# Autodesk Inventor assembly: 2020RobotV3
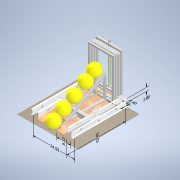
[picture p0: Inventor's stored thumbnail of the model, 180x180]
Saved by Autodesk Inventor 2020.2 (Build 242310000, 310)
## iProperties
Created: 2020-01-12
Part Number: 2020RobotV3
Document SubType Name: Assembly
Designer: robst
Author: robst
## Documents named in this file (15)
- C:\git\CAD-Development\robSteele\2020LongRobotBase\2020RobotV3.iam
- C:\git\CAD-Development\robSteele\2020LongRobotBase\2020 Wood Base.ipt
- C:\git\CAD-Development\robSteele\2020LongRobotBase\2020 End Plate.ipt
- C:\git\CAD-Development\robSteele\2020LongRobotBase\am-3921 AM14U4 Outside Plate.ipt
- C:\git\CAD-Development\robSteele\2020LongRobotBase\am-3922 AM14U4 Inside Plate.ipt
- C:\git\CAD-Development\robSteele\2020LongRobotBase\crossPlate.ipt
- C:\git\CAD-Development\robSteele\2020LongRobotBase\floor.ipt
- C:\git\CAD-Development\robSteele\2020LongRobotBase\1892-YEL.ipt
- C:\git\CAD-Development\robSteele\2020LongRobotBase\ceiling.ipt
- C:\git\CAD-Development\robSteele\2020LongRobotBase\asPrototypedBallRamp.iam
- C:\git\CAD-Development\robSteele\2020LongRobotBase\asPrototypedBallRamp_MIR.iam
- C:\git\CAD-Development\robSteele\2020LiftMechanism\primativeBaseForShortRobot.ipt
- C:\git\CAD-Development\robSteele\2020LiftMechanism\primative1stStageForShortRobot.ipt
- C:\git\CAD-Development\robSteele\2020LiftMechanism\primative4thStageForShortRobot.ipt
- C:\git\CAD-Development\robSteele\2020LiftMechanism\primative3rdStageForShortRobot.ipt
## Components (20 placed, 14 different names)
1. 2020 End Plate:1 — Mate:2, Mate:3, Mate:5, Mate:6, Flush:2, Flush:3, Mate:7, Mate:8, Mate:13, Mate:14, Mate:33, Flush:14, Mate:42, Mate:68
2. am-3921 AM14U4 Outside Plate:1 — Mate:5, Mate:6, Flush:2, Mate:15
3. am-3921 AM14U4 Outside Plate:2 — Mate:2, Mate:3, Flush:3, Mate:9
4. am-3922 AM14U4 Inside Plate:1 — Mate:7, Mate:8, Mate:9, Mate:12, Flush:4, Flush:5, Flush:12, Mate:32
5. crossPlate:1 — Mate:12, Flush:4, Flush:5
6. am-3922 AM14U4 Inside Plate:2 — Mate:13, Mate:14, Mate:15
7. floor:1 — Mate:54, Mate:55, Flush:18, Mate:65, Mate:66, Flush:30
8. 1892-YEL:1 — Mate:46, Mate:51
9. 1892-YEL:2 — Mate:50, Mate:52
10. 1892-YEL:3 — Mate:47, Mate:53
11. 1892-YEL:4 — Mate:48
12. 1892-YEL:5 — Mate:49
13. ceiling:1 — Mate:65, Mate:66, Flush:30
14. 2020 Wood Base:1 — Flush:13, Mate:32, Mate:33, Mate:35, Mate:37, Flush:16, Mate:39, Mate:54
15. asPrototypedBallRamp:1 [sub-assembly] — Mate:34, Mate:35, Flush:14, Flush:17
16. asPrototypedBallRamp_MIR:1 [sub-assembly] — Flush:15
17. primativeBaseForShortRobot:1 — Mate:36, Mate:37, Flush:16, Mate:40
18. primative1stStageForShortRobot:1 — Mate:38, Mate:39, Mate:40, Mate:43
19. primative3rdStageForShortRobot:1 — Mate:41, Mate:42, Mate:43, Mate:45
20. primative4thStageForShortRobot:1 — Mate:45, Mate:67, Mate:68
## Relationships (50: Mate 38, Flush 12)
- Mate:2: 2020 End Plate:1 ↔ am-3921 AM14U4 Outside Plate:2
- Mate:3 (30.48 mm): 2020 End Plate:1 ↔ am-3921 AM14U4 Outside Plate:2
- Mate:5: 2020 End Plate:1 ↔ am-3921 AM14U4 Outside Plate:1
- Mate:6 (30.48 mm): 2020 End Plate:1 ↔ am-3921 AM14U4 Outside Plate:1
- Flush:2: 2020 End Plate:1 ↔ am-3921 AM14U4 Outside Plate:1
- Flush:3: 2020 End Plate:1 ↔ am-3921 AM14U4 Outside Plate:2
- Mate:7: 2020 End Plate:1 ↔ am-3922 AM14U4 Inside Plate:1
- Mate:8 (30.48 mm): 2020 End Plate:1 ↔ am-3922 AM14U4 Inside Plate:1
- Mate:9 (85.725 mm): am-3921 AM14U4 Outside Plate:2 ↔ am-3922 AM14U4 Inside Plate:1
- Mate:12: am-3922 AM14U4 Inside Plate:1 ↔ crossPlate:1
- Flush:4: am-3922 AM14U4 Inside Plate:1 ↔ crossPlate:1
- Flush:5 (304.8 mm): am-3922 AM14U4 Inside Plate:1 ↔ crossPlate:1
- Mate:13: 2020 End Plate:1 ↔ am-3922 AM14U4 Inside Plate:2
- Mate:14: 2020 End Plate:1 ↔ am-3922 AM14U4 Inside Plate:2
- Mate:15 (85.725 mm): am-3921 AM14U4 Outside Plate:1 ↔ am-3922 AM14U4 Inside Plate:2
- Flush:12 (200.025 mm): am-3922 AM14U4 Inside Plate:1
- Flush:13: 2020 Wood Base:1
- Mate:32: am-3922 AM14U4 Inside Plate:1 ↔ 2020 Wood Base:1
- Mate:33: 2020 End Plate:1 ↔ 2020 Wood Base:1
- Mate:34 (57.15 mm): asPrototypedBallRamp:1
- Mate:35: 2020 Wood Base:1 ↔ asPrototypedBallRamp:1
- Flush:14 (114.935 mm): 2020 End Plate:1 ↔ asPrototypedBallRamp:1
- Flush:15 (57.15 mm): asPrototypedBallRamp_MIR:1
- Mate:36: primativeBaseForShortRobot:1
- Mate:37: 2020 Wood Base:1 ↔ primativeBaseForShortRobot:1
- Flush:16 (-88.9 mm): 2020 Wood Base:1 ↔ primativeBaseForShortRobot:1
- Mate:38: primative1stStageForShortRobot:1
- Mate:39: 2020 Wood Base:1 ↔ primative1stStageForShortRobot:1
- Mate:40 (12.7 mm): primativeBaseForShortRobot:1 ↔ primative1stStageForShortRobot:1
- Mate:41: primative3rdStageForShortRobot:1
- Mate:42: 2020 End Plate:1 ↔ primative3rdStageForShortRobot:1
- Mate:43 (12.7 mm): primative1stStageForShortRobot:1 ↔ primative3rdStageForShortRobot:1
- Mate:45 (12.7 mm): primative3rdStageForShortRobot:1 ↔ primative4thStageForShortRobot:1
- Flush:17 (76.2 mm): asPrototypedBallRamp:1
- Mate:46: 1892-YEL:1
- Mate:47: 1892-YEL:3
- Mate:48: 1892-YEL:4
- Mate:49: 1892-YEL:5
- Mate:50: 1892-YEL:2
- Mate:51: 1892-YEL:1
- Mate:52: 1892-YEL:2
- Mate:53: 1892-YEL:3
- Mate:54 (50.8 mm): floor:1 ↔ 2020 Wood Base:1
- Mate:55: floor:1
- Flush:18: floor:1
- Mate:65 (711.2 mm): floor:1 ↔ ceiling:1
- Mate:66: floor:1 ↔ ceiling:1
- Flush:30: floor:1 ↔ ceiling:1
- Mate:67: primative4thStageForShortRobot:1
- Mate:68: 2020 End Plate:1 ↔ primative4thStageForShortRobot:1
